# Autodesk Inventor assembly: VEX Claw Finger
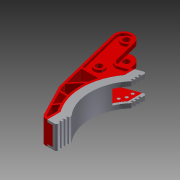
[picture p0: Inventor's stored thumbnail of the model, 180x180]
Saved by Autodesk Inventor 2013 (Build 170138000, 138)
## iProperties
Created: 2011-04-06
Part Number: VEX Claw Finger
Document SubType Name: Assembly
Designer: Phillip
Author: Phillip
## Documents named in this file (3)
- C:\Data Folder\VEX 2012\VEX KOP Uploads\2013\Metric\Motion\Components\VEX Claw Finger.iam
- C:\Data Folder\VEX 2012\VEX KOP Uploads\2013\Metric\Motion\Components\VEX Claw Finger.ipt
- C:\Data Folder\VEX 2012\VEX KOP Uploads\2013\Metric\Motion\Components\VEX Claw Gripper.ipt
## Components (2 placed, 2 different names)
1. VEX Claw Finger:1 — Flush:1, Flush:3, Mate:1
2. VEX Claw Gripper:1 — Flush:1, Flush:3, Mate:1
## Relationships (3: Flush 2, Mate 1)
- Flush:1: VEX Claw Finger:1 ↔ VEX Claw Gripper:1
- Flush:3: VEX Claw Finger:1 ↔ VEX Claw Gripper:1
- Mate:1: VEX Claw Finger:1 ↔ VEX Claw Gripper:1
